# Autodesk Inventor assembly: Elevator
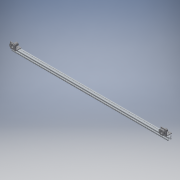
[picture p0: Inventor's stored thumbnail of the model, 180x180]
Saved by Autodesk Inventor 2017 (Build 210142000, 142)
## iProperties
Created: 2016-12-12
Part Number: Elevator
Document SubType Name: Assembly
Designer: umr
Mass: 2299.93 g
Surface Area: 5139.57 cm^2
Volume: 605.03 cm^3
Density: 3.80135 g/cm^3
Author: umr
## Documents named in this file (8)
- D:\SeniorProject\Models2\Gantry\GantryUp.iam
- D:\SeniorProject\Models2\Gantry\Tee Nut With headless screw.iam
- D:\SeniorProject\Models2\Gantry\HeaderTrack.ipt
- D:\SeniorProject\Models2\PowerScrewNut.ipt
- D:\SeniorProject\Models2\LBent_PScrew.ipt
- D:\SeniorProject\Models2\Gantry\Tee Nut With headless screw_MIR.iam
- D:\SeniorProject\Models2\PowerScrewNut_MIR.ipt
- D:\SeniorProject\Models2\LBent_PScrew_MIR.ipt
## Components (9 placed, 7 different names)
1. Tee Nut With headless screw:2 [sub-assembly] — Mate:79, Mate:80, Mate:85
2. HeaderTrack:1 — Mate:79, Mate:80, Mate:84, Mate:86, Flush:1
3. PowerScrewNut:1 — Mate:81, Mate:82, Mate:83
4. LBent_PScrew:1 — Mate:81, Mate:82, Mate:83, Mate:85, Mate:86, Mate:87, Flush:1
5. Tee Nut With headless screw:3 [sub-assembly] — Mate:84, Mate:87
6. Tee Nut With headless screw_MIR:1 [sub-assembly] — Mate:88
7. PowerScrewNut_MIR:1 — Mate:89, Mate:90, Mate:91
8. LBent_PScrew_MIR:1 — Mate:88, Mate:89, Mate:90, Mate:91, Mate:92
9. Tee Nut With headless screw_MIR:2 [sub-assembly] — Mate:92
## Relationships (15: Mate 14, Flush 1)
- Mate:79: Tee Nut With headless screw:2 ↔ HeaderTrack:1
- Mate:80: Tee Nut With headless screw:2 ↔ HeaderTrack:1
- Mate:81: PowerScrewNut:1 ↔ LBent_PScrew:1
- Mate:82: PowerScrewNut:1 ↔ LBent_PScrew:1
- Mate:83: PowerScrewNut:1 ↔ LBent_PScrew:1
- Mate:84: HeaderTrack:1 ↔ Tee Nut With headless screw:3
- Mate:85: Tee Nut With headless screw:2 ↔ LBent_PScrew:1
- Mate:86: HeaderTrack:1 ↔ LBent_PScrew:1
- Mate:87: LBent_PScrew:1 ↔ Tee Nut With headless screw:3
- Flush:1: HeaderTrack:1 ↔ LBent_PScrew:1
- Mate:88: Tee Nut With headless screw_MIR:1 ↔ LBent_PScrew_MIR:1
- Mate:89: PowerScrewNut_MIR:1 ↔ LBent_PScrew_MIR:1
- Mate:90: PowerScrewNut_MIR:1 ↔ LBent_PScrew_MIR:1
- Mate:91: PowerScrewNut_MIR:1 ↔ LBent_PScrew_MIR:1
- Mate:92: LBent_PScrew_MIR:1 ↔ Tee Nut With headless screw_MIR:2
